# Autodesk Inventor assembly: MotionBaseGeneric
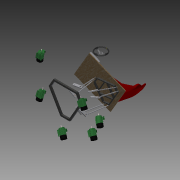
[picture p0: Inventor's stored thumbnail of the model, 180x180]
Saved by Autodesk Inventor 2015 SP1 (Build 190203100, 203)
## iProperties
Created: 2016-02-02
Part Number: MotionBaseGeneric
Document SubType Name: Assembly
Designer: tuttlem
Author: tuttlem
## Documents named in this file (14)
- C:\Users\jonesdm\Desktop\motionbase\CAD\MotionBaseCAD\MotionBaseGeneric.iam
- C:\Users\jonesdm\Desktop\motionbase\CAD\MotionBaseCAD\Platform.ipt
- C:\Users\jonesdm\Desktop\motionbase\CAD\MotionBaseCAD\BasePlatform.ipt
- C:\Users\jonesdm\Desktop\motionbase\CAD\MotionBaseCAD\Rod.ipt
- C:\Users\jonesdm\Desktop\motionbase\CAD\MotionBaseCAD\Rod_MIR.ipt
- C:\Users\jonesdm\Desktop\motionbase\CAD\MotionBaseCAD\arm.ipt
- C:\Users\jonesdm\Desktop\motionbase\CAD\MotionBaseCAD\Bearing.ipt
- C:\Users\jonesdm\Desktop\motionbase\CAD\MotionBaseCAD\siege.ipt
- C:\Users\jonesdm\Desktop\motionbase\CAD\MotionBaseCAD\Sparco Volante wheel.ipt
- C:\Users\jonesdm\Desktop\motionbase\CAD\MotionBaseCAD\TopPlatform.ipt
- C:\Users\jonesdm\Documents\Inventor\00 - Pedalier CSP V2.iam
- C:\Users\jonesdm\Desktop\motionbase\CAD\MotionBaseCAD\Side Rail.ipt
- C:\Users\jonesdm\Desktop\motionbase\CAD\MotionBaseCAD\Front Rail.ipt
- C:\Users\jonesdm\Desktop\motionbase\CAD\MotionBaseCAD\Motor3.ipt
## Components (40 placed, 13 different names)
1. Platform:1 — Insert:3, Insert:5, Mate:1, Flush:7, Mate:2, Flush:8, Mate:3, Mate:4, Mate:5, Flush:9, Wood To Metal, Wood To Back, Mate:66
2. BasePlatform:1 — Mate:6, Angle:1, Mate:71
3. seat — Seat To Wood, Seat To Back, Seat Centered, Angle:9, Mate:72
4. Sparco Volante wheel:1
5. TopPlatform:1 — Wood To Metal, Wood To Back, Angle:8, Seat To Left, Seat To Wood, Seat To Back, Seat Centered, Pedals to Wood, Pedals to Front, Pedals to Center, Mate:75, Mate:76, Flush:24, Flush:25, Flush:26, Flush:27, Mate:77, Flush:29, Flush:30, Mate:78, Flush:31, Flush:32
6. 00 - Pedalier CSP V2:1 [sub-assembly] — Pedals to Wood, Pedals to Front, Pedals to Center
7. Side Rail:1 — Mate:75, Flush:24, Flush:26
8. Side Rail:2 — Mate:76, Flush:25, Flush:27
9. Front Rail:1 — Mate:77, Flush:29, Flush:30
10. Front Rail:2 — Mate:78, Flush:31, Flush:32
11. Motor3:1
12. Motor3:2
13. Motor3:3
14. Motor3:4
15. Motor3:5
16. Motor3:6
17. Rod_MIR:1 — Flush:1, Tangent:1, Mate:40
18. Rod_MIR:2 — Mate:31
19. Rod_MIR:3 — Mate:28
20. Rod_MIR:4 — Mate:29
21. Rod_MIR:5 — Mate:60
22. Rod_MIR:6 — Mate:32
23. Rod:1 — Flush:1, Tangent:1, Insert:3
24. Rod:2 — Insert:5
25. Rod:3 — Mate:1, Flush:7
26. Rod:4 — Mate:2, Flush:8
27. Rod:5 — Mate:3, Mate:4
28. Rod:6 — Mate:5, Flush:9
29. arm:1 — Mate:43
30. arm:8 — Mate:63
31. arm:9 — Mate:42
32. arm:10 — Mate:61
33. arm:11 — Mate:62
34. arm:12 — Mate:64
35. Bearing:2 — Mate:40, Mate:64
36. Bearing:3 — Mate:60, Mate:61
37. Bearing:4 — Mate:32, Mate:62
38. Bearing:5 — Mate:29, Mate:43
39. Bearing:6 — Mate:28, Mate:42
40. Bearing:1 — Mate:31, Mate:63
## Relationships (65: Mate 30, Flush 22, Tangent 6, Angle 5, Insert 2)
- Flush:1: Rod_MIR:1 ↔ Rod:1
- Tangent:1: Rod_MIR:1 ↔ Rod:1
- [Flush]: Rod_MIR:2 ↔ Rod:2
- [Tangent]: Rod_MIR:2 ↔ Rod:2
- Insert:3: Platform:1 ↔ Rod:1
- Insert:5: Platform:1 ↔ Rod:2
- [Flush]: Rod_MIR:3 ↔ Rod:3
- [Tangent]: Rod_MIR:3 ↔ Rod:3
- [Flush]: Rod_MIR:4 ↔ Rod:4
- [Tangent]: Rod_MIR:4 ↔ Rod:4
- [Flush]: Rod_MIR:5 ↔ Rod:5
- [Tangent]: Rod_MIR:5 ↔ Rod:5
- [Flush]: Rod_MIR:6 ↔ Rod:6
- [Tangent]: Rod_MIR:6 ↔ Rod:6
- Mate:1: Platform:1 ↔ Rod:3
- Flush:7: Platform:1 ↔ Rod:3
- Mate:2: Platform:1 ↔ Rod:4
- Flush:8: Platform:1 ↔ Rod:4
- Mate:3: Platform:1 ↔ Rod:5
- Mate:4: Platform:1 ↔ Rod:5
- Mate:5: Platform:1 ↔ Rod:6
- Flush:9: Platform:1 ↔ Rod:6
- Mate:6: BasePlatform:1
- Flush:10 (25.4 mm)
- Mate:28: Rod_MIR:3 ↔ Bearing:6
- Mate:29: Rod_MIR:4 ↔ Bearing:5
- Mate:31: Rod_MIR:2 ↔ Bearing:1
- Mate:32: Rod_MIR:6 ↔ Bearing:4
- Mate:40: Rod_MIR:1 ↔ Bearing:2
- Angle:1 (0 deg): BasePlatform:1
- Mate:42: arm:9 ↔ Bearing:6
- Mate:43: arm:1 ↔ Bearing:5
- Angle:5 (0 deg)
- Angle:7 (0 deg)
- Mate:60: Rod_MIR:5 ↔ Bearing:3
- Mate:61: arm:10 ↔ Bearing:3
- Mate:62: arm:11 ↔ Bearing:4
- Mate:63: arm:8 ↔ Bearing:1
- Mate:64: arm:12 ↔ Bearing:2
- Wood To Metal [Mate]: Platform:1 ↔ TopPlatform:1
- Wood To Back [Flush] (-101.6 mm): Platform:1 ↔ TopPlatform:1
- Mate:66: Platform:1
- Angle:8 (0 deg): TopPlatform:1
- Seat To Left [Flush] (-101.6 mm): TopPlatform:1
- Seat To Wood [Mate]: seat ↔ TopPlatform:1
- Seat To Back [Flush] (-76.2 mm): seat ↔ TopPlatform:1
- Seat Centered [Mate]: seat ↔ TopPlatform:1
- Mate:71: BasePlatform:1
- Angle:9 (0 deg): seat
- Mate:72: seat
- Pedals to Wood [Mate]: TopPlatform:1 ↔ 00 - Pedalier CSP V2:1
- Pedals to Front [Flush] (38.1 mm): TopPlatform:1 ↔ 00 - Pedalier CSP V2:1
- Pedals to Center [Mate] (25.4 mm): TopPlatform:1 ↔ 00 - Pedalier CSP V2:1
- Mate:75: TopPlatform:1 ↔ Side Rail:1
- Mate:76: TopPlatform:1 ↔ Side Rail:2
- Flush:24: TopPlatform:1 ↔ Side Rail:1
- Flush:25: TopPlatform:1 ↔ Side Rail:2
- Flush:26: TopPlatform:1 ↔ Side Rail:1
- Flush:27: TopPlatform:1 ↔ Side Rail:2
- Mate:77: TopPlatform:1 ↔ Front Rail:1
- Flush:29: TopPlatform:1 ↔ Front Rail:1
- Flush:30: TopPlatform:1 ↔ Front Rail:1
- Mate:78: TopPlatform:1 ↔ Front Rail:2
- Flush:31: TopPlatform:1 ↔ Front Rail:2
- Flush:32: TopPlatform:1 ↔ Front Rail:2
## Named parameters: d2_d1 = 0 mm, d3_d0 = 0 mm, d18_d1 = 0 mm, d21_d0 = 0 mm, d22_d1 = 0 mm, d25_d0 = 0 mm, d26_d1 = 0 mm, d29_d0 = 0 mm, d30_d1 = 0 mm, d33_d0 = 0 mm
